# Autodesk Inventor assembly: GE-13026
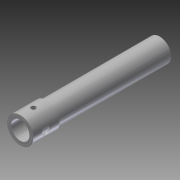
[picture p0: Inventor's stored thumbnail of the model, 180x180]
Saved by Autodesk Inventor 2013 (Build 170138000, 138)
## iProperties
Created: 2013-01-06
Part Number: GE-13026
Document SubType Name: Assembly
Designer: Phillip
Author: Phillip
## Documents named in this file (3)
- C:\Users\Moses\Documents\Inventor\2013 Team 3061 Robot\FIRST Arena 2013\Pyramid\GE-13026.iam
- C:\Users\Moses\Documents\Inventor\2013 Team 3061 Robot\FIRST Arena 2013\Pyramid\GE-13026-01.ipt
- C:\Users\Moses\Documents\Inventor\2013 Team 3061 Robot\FIRST Arena 2013\Pyramid\GE-13026-02.ipt
## Components (2 placed, 2 different names)
1. GE-13026-01:1 — Insert:1
2. GE-13026-02:1 — Insert:1
## Relationships (1: Insert 1)
- Insert:1: GE-13026-01:1 ↔ GE-13026-02:1
